# Autodesk Inventor assembly: Prezent_zlozony
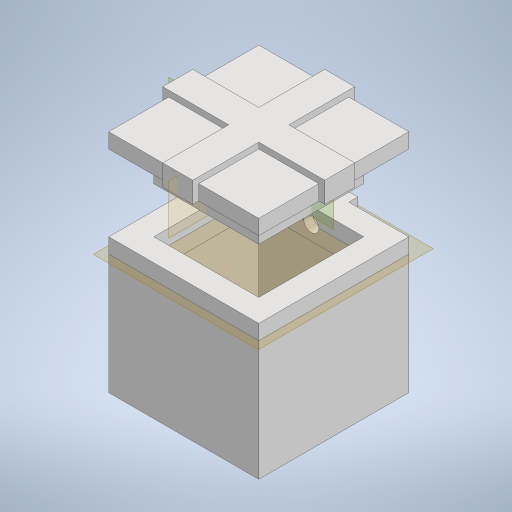
[picture p0: Inventor's stored thumbnail of the model, 512x512]
Saved by Autodesk Inventor 2024 (Build 280153000, 153)
## iProperties
Created: 2023-10-17
Part Number: Prezent_zlozony
Document SubType Name: Assembly
Designer: Piter
Author: Piter
## Documents named in this file (3)
- C:\Users\Piter\OneDrive\Pulpit\Modele\My projects\My-3D-printing-projects\Prezent\Prezent_zlozony.iam
- C:\Users\Piter\OneDrive\Pulpit\Modele\My projects\My-3D-printing-projects\Prezent\Pokrywka.ipt
- C:\Users\Piter\OneDrive\Pulpit\Modele\My projects\My-3D-printing-projects\Prezent\Pudelko.ipt
## Components (2 placed, 2 different names)
1. Pokrywka:1 — Mate:1, Mate:2
2. Pudelko:1 — Mate:1, Mate:2
## Relationships (2: Mate 2)
- Mate:1: Pokrywka:1 ↔ Pudelko:1
- Mate:2: Pokrywka:1 ↔ Pudelko:1
